# Autodesk Inventor assembly: assembledwheel
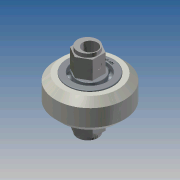
[picture p0: Inventor's stored thumbnail of the model, 180x180]
Saved by Autodesk Inventor 2015 (Build 190159000, 159)
## iProperties
Created: 2015-10-03
Part Number: assembledwheel
Document SubType Name: Assembly
Designer: Solomon
Author: Solomon
## Documents named in this file (4)
- C:\Users\Solomon\Documents\Inventor\Omni 1\V Slot Part Files\assembledwheel.iam
- C:\Users\Solomon\Documents\Inventor\Omni 1\Imported Components\5mm Bearing SKF 625 (RS 286-7811)\5mm Bearing SKF 625 (RS 286-7811).ipt
- C:\Users\Solomon\Documents\Inventor\Omni 1\V Slot Part Files\Pulleys Wheels Bearings\Solid V Wheel.ipt
- C:\Users\Solomon\Documents\Inventor\Omni 1\V Slot Part Files\Spacers\Eccentric M5 Spacer.ipt
## Components (5 placed, 3 different names)
1. 5mm Bearing SKF 625 (RS 286-7811):1 — Angle:1, Mate:1, Angle:2, Mate:4
2. Solid V Wheel:1 — Angle:1, Mate:1, Mate:2
3. 5mm Bearing SKF 625 (RS 286-7811):2 — Mate:2, Mate:3
4. Eccentric M5 Spacer:1 — Mate:3
5. Eccentric M5 Spacer:2 — Angle:2, Mate:4
## Relationships (6: Mate 4, Angle 2)
- Angle:1 (0 deg): 5mm Bearing SKF 625 (RS 286-7811):1 ↔ Solid V Wheel:1
- Mate:1: 5mm Bearing SKF 625 (RS 286-7811):1 ↔ Solid V Wheel:1
- Mate:2: Solid V Wheel:1 ↔ 5mm Bearing SKF 625 (RS 286-7811):2
- Mate:3: 5mm Bearing SKF 625 (RS 286-7811):2 ↔ Eccentric M5 Spacer:1
- Angle:2 (180 deg): 5mm Bearing SKF 625 (RS 286-7811):1 ↔ Eccentric M5 Spacer:2
- Mate:4: 5mm Bearing SKF 625 (RS 286-7811):1 ↔ Eccentric M5 Spacer:2
